# Autodesk Inventor assembly: Inner_Components
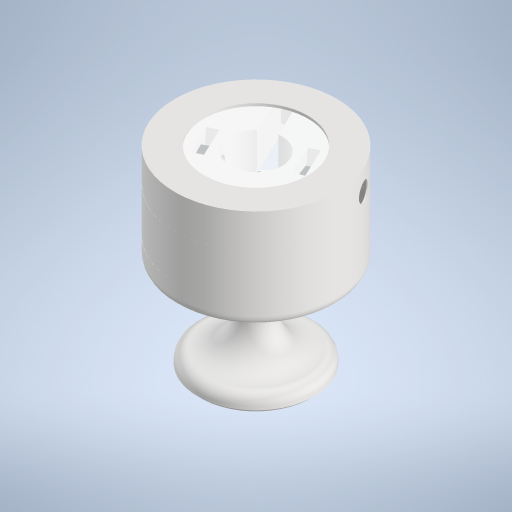
[picture p0: Inventor's stored thumbnail of the model, 512x512]
Saved by Autodesk Inventor 2023 (Build 270158000, 158)
## iProperties
Created: 2023-02-27
Part Number: Inner_Components
Document SubType Name: Assembly
Designer: maste
Author: maste
## Documents named in this file (8)
- C:\Users\maste\Documents\GitHub\Remote-Stethoscope\3D_models\ThonkLabs 1ne\SurfaceContact\Inner_Components.iam
- C:\Users\maste\Documents\GitHub\Remote-Stethoscope\3D_models\ThonkLabs 1ne\SurfaceContact\PiezoMount.ipt
- C:\Users\maste\Documents\GitHub\Remote-Stethoscope\3D_models\ThonkLabs 1ne\SurfaceContact\Diaphragm_lock.ipt
- C:\Users\maste\Documents\GitHub\Remote-Stethoscope\3D_models\ThonkLabs 1ne\SurfaceContact\holding_socket.ipt
- C:\Users\maste\Documents\GitHub\Remote-Stethoscope\3D_models\ThonkLabs 1ne\SurfaceContact\fasten_nut.ipt
- C:\Users\maste\Documents\GitHub\Remote-Stethoscope\3D_models\ThonkLabs 1ne\SurfaceContact\fasten_bolt.ipt
- C:\Users\maste\Documents\GitHub\Remote-Stethoscope\3D_models\ThonkLabs 1ne\SeparateDiaphragm\Diaphragm.ipt
- C:\Users\maste\Documents\GitHub\Remote-Stethoscope\3D_models\ThonkLabs 1ne\SeparateDiaphragm\CircuitCell.iam
## Components (13 placed, 7 different names)
1. PiezoMount:1 — Mate:7, Mate:8, Mate:10, Mate:14, Mate:16, Mate:23, Mate:24, Mate:25, Mate:28, Mate:31, Mate:32, Mate:36, Mate:37, Mate:38, Flush:2, Mate:43, Mate:44, Mate:45, Mate:46, Mate:47
2. Diaphragm_lock:1 — Mate:38, Mate:39
3. holding_socket:1 — Mate:7, Mate:8, Mate:10, Mate:18, Mate:19, Mate:20, Mate:21
4. fasten_nut:1 — Mate:14, Mate:23
5. fasten_nut:2 — Mate:16, Mate:24
6. fasten_bolt:1 — Mate:18, Mate:20
7. fasten_bolt:2 — Mate:19, Mate:21
8. fasten_nut:3 — Mate:28, Mate:41
9. fasten_nut:4 — Mate:25, Mate:42
10. fasten_bolt:3 — Mate:31, Mate:42, Mate:46
11. fasten_bolt:4 — Mate:32, Mate:41, Mate:47
12. Diaphragm:1 — Mate:36, Mate:37, Mate:39
13. CircuitCell:1 [sub-assembly] — Mate:43, Mate:44, Mate:45
## Relationships (27: Mate 26, Flush 1)
- Mate:7: PiezoMount:1 ↔ holding_socket:1
- Mate:8: PiezoMount:1 ↔ holding_socket:1
- Mate:10: PiezoMount:1 ↔ holding_socket:1
- Mate:14: PiezoMount:1 ↔ fasten_nut:1
- Mate:16: PiezoMount:1 ↔ fasten_nut:2
- Mate:18: holding_socket:1 ↔ fasten_bolt:1
- Mate:19: holding_socket:1 ↔ fasten_bolt:2
- Mate:20: holding_socket:1 ↔ fasten_bolt:1
- Mate:21: holding_socket:1 ↔ fasten_bolt:2
- Mate:23: PiezoMount:1 ↔ fasten_nut:1
- Mate:24: PiezoMount:1 ↔ fasten_nut:2
- Mate:25: PiezoMount:1 ↔ fasten_nut:4
- Mate:28: PiezoMount:1 ↔ fasten_nut:3
- Mate:31: PiezoMount:1 ↔ fasten_bolt:3
- Mate:32: PiezoMount:1 ↔ fasten_bolt:4
- Mate:36: PiezoMount:1 ↔ Diaphragm:1
- Mate:37: PiezoMount:1 ↔ Diaphragm:1
- Mate:38: PiezoMount:1 ↔ Diaphragm_lock:1
- Mate:39: Diaphragm_lock:1 ↔ Diaphragm:1
- Flush:2 (33 mm): PiezoMount:1
- Mate:41: fasten_nut:3 ↔ fasten_bolt:4
- Mate:42: fasten_nut:4 ↔ fasten_bolt:3
- Mate:43: PiezoMount:1 ↔ CircuitCell:1
- Mate:44: PiezoMount:1 ↔ CircuitCell:1
- Mate:45 (1 mm): PiezoMount:1 ↔ CircuitCell:1
- Mate:46: PiezoMount:1 ↔ fasten_bolt:3
- Mate:47: PiezoMount:1 ↔ fasten_bolt:4
